# Autodesk Inventor assembly: 二段_多段ギア
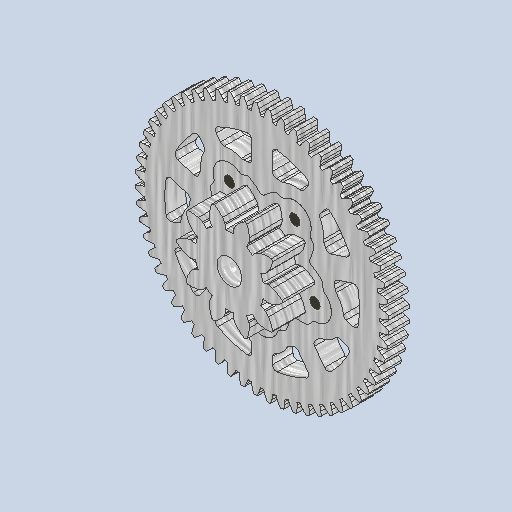
[picture p0: Inventor's stored thumbnail of the model, 512x512]
Saved by Autodesk Inventor 2023 (Build 270158030, 158C)
## iProperties
Created: 2022-06-25
Part Number: 二段_多段ギア
Document SubType Name: Assembly
Designer: muzho
Author: muzho
## Documents named in this file (4)
- C:\Users\muzho\Documents\srdc\srdc_2\アーム\ギア\二段_多段ギア.iam
- C:\Users\muzho\Documents\srdc\srdc_2\アーム\ギア\二段m1z60.ipt
- C:\Users\muzho\Documents\srdc\srdc_2\アーム\ギア\m2z10t8.ipt
- C:\Users\muzho\Documents\srdc\srdc_2\ねじ\SB　5mm皿ネジ.ipt
## Components (7 placed, 3 different names)
1. 二段m1z60:1 — メイト:1, メイト:2, メイト:3, 挿入:1, 挿入:2, 挿入:3, 挿入:4, 挿入:5, 挿入:6
2. m2z10t8:1 — メイト:1, メイト:2, メイト:3, 挿入:1
3. SB　5mm皿ネジ:1 — 挿入:2
4. SB　5mm皿ネジ:2 — 挿入:3
5. SB　5mm皿ネジ:3 — 挿入:4
6. SB　5mm皿ネジ:4 — 挿入:6
7. SB　5mm皿ネジ:5 — 挿入:5
## Relationships (9: Insert 6, Mate 3)
- メイト:1 [Mate]: 二段m1z60:1 ↔ m2z10t8:1
- メイト:2 [Mate]: 二段m1z60:1 ↔ m2z10t8:1
- メイト:3 [Mate]: 二段m1z60:1 ↔ m2z10t8:1
- 挿入:1 [Insert]: 二段m1z60:1 ↔ m2z10t8:1
- 挿入:2 [Insert]: 二段m1z60:1 ↔ SB　5mm皿ネジ:1
- 挿入:3 [Insert]: 二段m1z60:1 ↔ SB　5mm皿ネジ:2
- 挿入:4 [Insert]: 二段m1z60:1 ↔ SB　5mm皿ネジ:3
- 挿入:5 [Insert]: 二段m1z60:1 ↔ SB　5mm皿ネジ:5
- 挿入:6 [Insert]: 二段m1z60:1 ↔ SB　5mm皿ネジ:4
